# Autodesk Inventor assembly: door assembly for 2nd map
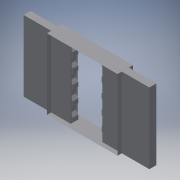
[picture p0: Inventor's stored thumbnail of the model, 180x180]
Saved by Autodesk Inventor 2017 (Build 210142000, 142)
## iProperties
Created: 2018-05-21
Part Number: door assembly for 2nd map
Document SubType Name: Assembly
Designer: braxtonwright
Author: braxtonwright
## Documents named in this file (4)
- D:\School\Game develpment\geoscape\doors\assembly\door assembly for 2nd map.iam
- D:\School\Game develpment\geoscape\doors\doorframe 2nd map.ipt
- D:\School\Game develpment\geoscape\doors\door (right side) 2nd map.ipt
- D:\School\Game develpment\geoscape\doors\door (left side) 2nd map.ipt
## Components (3 placed, 3 different names)
1. doorframe 2nd map:1 — Mate:1, Mate:2, Flush:1, Mate:3, Mate:4, Flush:2
2. door (right side) 2nd map:1 — Mate:1, Mate:2, Flush:1
3. door (left side) 2nd map:1 — Mate:3, Mate:4, Flush:2
## Relationships (6: Mate 4, Flush 2)
- Mate:1: doorframe 2nd map:1 ↔ door (right side) 2nd map:1
- Mate:2: doorframe 2nd map:1 ↔ door (right side) 2nd map:1
- Flush:1 (-63.5 mm): doorframe 2nd map:1 ↔ door (right side) 2nd map:1
- Mate:3: doorframe 2nd map:1 ↔ door (left side) 2nd map:1
- Mate:4: doorframe 2nd map:1 ↔ door (left side) 2nd map:1
- Flush:2 (-63.5 mm): doorframe 2nd map:1 ↔ door (left side) 2nd map:1
